# Autodesk Inventor assembly: LargeHubShaftServoBlock(24T Spline)-1111-2017
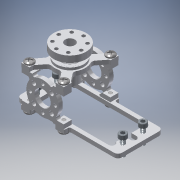
[picture p0: Inventor's stored thumbnail of the model, 180x180]
Saved by Autodesk Inventor 2016 SP2 (Build 200236200, 236)
## iProperties
Created: 2017-02-17
Part Number: LargeHubShaftServoBlock(24T Spline)-1111-2017
Document SubType Name: Assembly
Designer: 589013
Mass: 46.2322 g
Surface Area: 171.456 cm^2
Volume: 14.2987 cm^3
Density: 3.23332 g/cm^3
Author: 589013
## Documents named in this file (7)
- E:\GrabCAD\Power Hawks CAD\ServoCity Resources\Servo Mount\LargeHubShaftServoBlock(24T Spline)-1111-2017.iam
- E:\GrabCAD\Power Hawks CAD\ServoCity Resources\Servo Mount\Large Hub Shaft ServoBlock (24T Spline)\ServoPlate(637118)-1111-2017.ipt
- E:\GrabCAD\Power Hawks CAD\ServoCity Resources\Servo Mount\Large Hub Shaft ServoBlock (24T Spline)\HubPlate(637118)-1111-2017.ipt
- E:\GrabCAD\Power Hawks CAD\ServoCity Resources\Servo Mount\Large Hub Shaft ServoBlock (24T Spline)\BallBearingPlate(637118)-1111-2017.ipt
- E:\GrabCAD\Power Hawks CAD\ServoCity Resources\Servo Mount\Large Hub Shaft ServoBlock (24T Spline)\6-32Screw(637118)-1111-2017.ipt
- E:\GrabCAD\Power Hawks CAD\ServoCity Resources\Servo Mount\Large Hub Shaft ServoBlock (24T Spline)\ServoSplineShaftHub(637118)-1111-2017.ipt
- E:\GrabCAD\Power Hawks CAD\ServoCity Resources\Fasteners\6-32ZincPlatedSocketHeadMachineScrews-1111-2017.ipt
## Components (17 placed, 6 different names)
1. ServoPlate(637118)-1111-2017:1 — Rigid:1, Rigid:2, Rotational:5, Rotational:6, Rotational:7, Rotational:8, Insert:1, Insert:2, Insert:3, Insert:4
2. HubPlate(637118)-1111-2017:1 — Rigid:2
3. HubPlate(637118)-1111-2017:2 — Rigid:1, Rigid:3
4. BallBearingPlate(637118)-1111-2017:1 — Rotational:1, Rotational:2, Rotational:4, Cylindrical:10, Flush:1, Rigid:3, Rotational:9
5. ServoSplineShaftHub(637118)-1111-2017:1 — Cylindrical:10, Flush:1
6. 6-32Screw(637118)-1111-2017:9 — Rotational:9
7. 6-32ZincPlatedSocketHeadMachineScrews-1111-2017:1 — Insert:3
8. 6-32ZincPlatedSocketHeadMachineScrews-1111-2017:2 — Insert:4
9. 6-32ZincPlatedSocketHeadMachineScrews-1111-2017:3 — Insert:1
10. 6-32ZincPlatedSocketHeadMachineScrews-1111-2017:4 — Insert:2
11. 6-32Screw(637118)-1111-2017:2 — Rotational:1
12. 6-32Screw(637118)-1111-2017:3 — Rotational:4
13. 6-32Screw(637118)-1111-2017:4 — Rotational:2
14. 6-32Screw(637118)-1111-2017:5 — Rotational:5
15. 6-32Screw(637118)-1111-2017:6 — Rotational:8
16. 6-32Screw(637118)-1111-2017:7 — Rotational:6
17. 6-32Screw(637118)-1111-2017:8 — Rotational:7
## Relationships (17: RevoluteJoint 8, Insert 4, WeldJoint 3, CylindricalJoint 1, Flush 1)
- Rigid:1 [WeldJoint]: ServoPlate(637118)-1111-2017:1 ↔ HubPlate(637118)-1111-2017:2
- Rigid:2 [WeldJoint]: ServoPlate(637118)-1111-2017:1 ↔ HubPlate(637118)-1111-2017:1
- Rotational:1 [RevoluteJoint]: BallBearingPlate(637118)-1111-2017:1 ↔ 6-32Screw(637118)-1111-2017:2
- Rotational:2 [RevoluteJoint]: BallBearingPlate(637118)-1111-2017:1 ↔ 6-32Screw(637118)-1111-2017:4
- Rotational:4 [RevoluteJoint]: BallBearingPlate(637118)-1111-2017:1 ↔ 6-32Screw(637118)-1111-2017:3
- Rotational:5 [RevoluteJoint]: ServoPlate(637118)-1111-2017:1 ↔ 6-32Screw(637118)-1111-2017:5
- Rotational:6 [RevoluteJoint]: ServoPlate(637118)-1111-2017:1 ↔ 6-32Screw(637118)-1111-2017:7
- Rotational:7 [RevoluteJoint]: ServoPlate(637118)-1111-2017:1 ↔ 6-32Screw(637118)-1111-2017:8
- Rotational:8 [RevoluteJoint]: ServoPlate(637118)-1111-2017:1 ↔ 6-32Screw(637118)-1111-2017:6
- Cylindrical:10: BallBearingPlate(637118)-1111-2017:1 ↔ ServoSplineShaftHub(637118)-1111-2017:1
- Flush:1 (-11.43 mm): BallBearingPlate(637118)-1111-2017:1 ↔ ServoSplineShaftHub(637118)-1111-2017:1
- Insert:1 (3.81 mm): ServoPlate(637118)-1111-2017:1 ↔ 6-32ZincPlatedSocketHeadMachineScrews-1111-2017:3
- Insert:2 (3.81 mm): ServoPlate(637118)-1111-2017:1 ↔ 6-32ZincPlatedSocketHeadMachineScrews-1111-2017:4
- Insert:3 (3.81 mm): ServoPlate(637118)-1111-2017:1 ↔ 6-32ZincPlatedSocketHeadMachineScrews-1111-2017:1
- Insert:4 (3.81 mm): ServoPlate(637118)-1111-2017:1 ↔ 6-32ZincPlatedSocketHeadMachineScrews-1111-2017:2
- Rigid:3 [WeldJoint]: HubPlate(637118)-1111-2017:2 ↔ BallBearingPlate(637118)-1111-2017:1
- Rotational:9 [RevoluteJoint]: BallBearingPlate(637118)-1111-2017:1 ↔ 6-32Screw(637118)-1111-2017:9
